# Autodesk Inventor assembly: arm_test
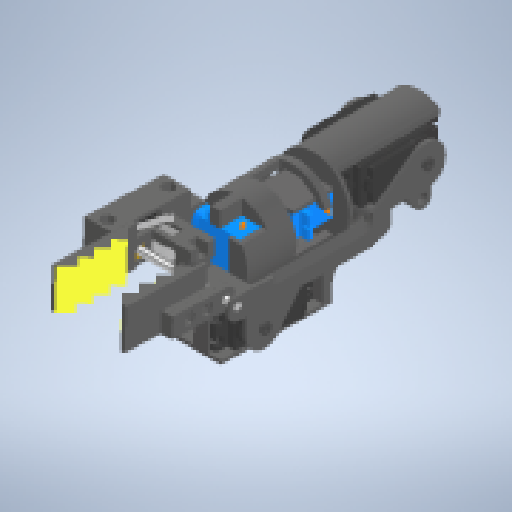
[picture p0: Inventor's stored thumbnail of the model, 512x512]
Saved by Autodesk Inventor 2024.1 (Build 281209000, 209)
## iProperties
Created: 2025-01-27
Part Number: arm_test
Document SubType Name: Assembly
Designer: hibik
Author: hibik
## Documents named in this file (15)
- C:\Users\hibik\Documents\Robomech\RESCUE\ORCA\hard\arm\arm_test.iam
- C:\Users\hibik\Documents\Robomech\RESCUE\ORCA\hard\arm\wrist_wrist.ipt
- C:\Users\hibik\Documents\Robomech\RESCUE\ORCA\hard\std_parts\Miusei_ms18.ipt
- C:\Users\hibik\Documents\Robomech\RESCUE\ORCA\hard\arm\wrist_geard_hone.ipt
- C:\Users\hibik\Documents\Robomech\RESCUE\ORCA\hard\arm\arm_2.ipt
- C:\Users\hibik\Documents\Robomech\RESCUE\ORCA\hard\std_parts\FS5103B.ipt
- C:\Users\hibik\Documents\Robomech\RESCUE\ORCA\hard\arm\arm_1.ipt
- C:\Users\hibik\Documents\Robomech\RESCUE\ORCA\hard\arm\hand_motor_setter_base.ipt
- C:\Users\hibik\Documents\Robomech\RESCUE\ORCA\hard\std_parts\motor_M4_55.ipt
- C:\Users\hibik\Documents\Robomech\RESCUE\ORCA\hard\std_parts\limit_switch.ipt
- C:\Users\hibik\Documents\Robomech\RESCUE\ORCA\hard\arm\hand_finger_inside.ipt
- C:\Users\hibik\Documents\Robomech\RESCUE\ORCA\hard\arm\hand_finger_outside.ipt
- C:\Users\hibik\Documents\Robomech\RESCUE\ORCA\hard\arm\hand_motor_setter_cover_under.ipt
- C:\Users\hibik\Documents\Robomech\RESCUE\ORCA\hard\arm\arm_0.ipt
- C:\Users\hibik\Documents\Robomech\RESCUE\ORCA\hard\arm\finger.ipt
## Components (17 placed, 14 different names)
1. wrist_wrist:1 — メイト:1, メイト:2, メイト:3, フラッシュ:2, メイト:4
2. Miusei_ms18:1 — メイト:1, メイト:2, メイト:3, フラッシュ:1, 挿入:3
3. Miusei_ms18:2 — 挿入:1, フラッシュ:1, フラッシュ:2, メイト:4, メイト:5, フラッシュ:3, フラッシュ:4
4. wrist_geard_hone:1 — 挿入:1
5. arm_2:1 — メイト:5, フラッシュ:3, フラッシュ:4, メイト:7, メイト:8, メイト:9
6. FS5103B:1 — メイト:7, メイト:8, 挿入:2, メイト:9
7. arm_1:1 — 挿入:2, 挿入:10
8. hand_motor_setter_base:1 — 挿入:3, 挿入:4, 角度:1, 挿入:5, 挿入:6, 角度:3, 角度:4, 挿入:8, 挿入:9, メイト:13, フラッシュ:5, メイト:14
9. motor_M4_55:1 — 挿入:4, 角度:1, 正接:1
10. limit_switch:1 — 挿入:5, 挿入:6
11. hand_finger_inside:1 — 挿入:7, 角度:2, 正接:1, 角度:4
12. hand_finger_outside:1 — 挿入:7, 角度:2, 角度:3, メイト:15
13. hand_motor_setter_cover_under:1 — 挿入:8, 挿入:9
14. arm_0:1 — メイト:10, メイト:11, メイト:12
15. FS5103B:2 — メイト:10, メイト:11, メイト:12, 挿入:10
16. finger:1 — メイト:13, フラッシュ:5, メイト:14, フラッシュ:6, フラッシュ:7
17. finger:2 — メイト:15, フラッシュ:6, フラッシュ:7
## Relationships (36: Mate 14, Insert 10, Flush 7, Angle 4, Tangent 1)
- メイト:1 [Mate]: wrist_wrist:1 ↔ Miusei_ms18:1
- メイト:2 [Mate]: wrist_wrist:1 ↔ Miusei_ms18:1
- メイト:3 [Mate] (0.1 mm): wrist_wrist:1 ↔ Miusei_ms18:1
- 挿入:1 [Insert]: Miusei_ms18:2 ↔ wrist_geard_hone:1
- フラッシュ:1 [Flush] (5.15 mm): Miusei_ms18:1 ↔ Miusei_ms18:2
- フラッシュ:2 [Flush] (-8 mm): wrist_wrist:1 ↔ Miusei_ms18:2
- メイト:4 [Mate] (2.4 mm): wrist_wrist:1 ↔ Miusei_ms18:2
- メイト:5 [Mate]: Miusei_ms18:2 ↔ arm_2:1
- フラッシュ:3 [Flush]: Miusei_ms18:2 ↔ arm_2:1
- フラッシュ:4 [Flush]: Miusei_ms18:2 ↔ arm_2:1
- メイト:7 [Mate]: arm_2:1 ↔ FS5103B:1
- メイト:8 [Mate]: arm_2:1 ↔ FS5103B:1
- 挿入:2 [Insert]: FS5103B:1 ↔ arm_1:1
- メイト:9 [Mate]: arm_2:1 ↔ FS5103B:1
- 挿入:3 [Insert]: Miusei_ms18:1 ↔ hand_motor_setter_base:1
- 挿入:4 [Insert] (0.1 mm): hand_motor_setter_base:1 ↔ motor_M4_55:1
- 角度:1 [Angle] (0 deg): hand_motor_setter_base:1 ↔ motor_M4_55:1
- 挿入:5 [Insert]: hand_motor_setter_base:1 ↔ limit_switch:1
- 挿入:6 [Insert]: hand_motor_setter_base:1 ↔ limit_switch:1
- 挿入:7 [Insert]: hand_finger_inside:1 ↔ hand_finger_outside:1
- 角度:2 [Angle] (180 deg): hand_finger_inside:1 ↔ hand_finger_outside:1
- 正接:1 [Tangent]: motor_M4_55:1 ↔ hand_finger_inside:1
- 角度:3 [Angle] (0 deg): hand_motor_setter_base:1 ↔ hand_finger_outside:1
- 角度:4 [Angle] (0 deg): hand_motor_setter_base:1 ↔ hand_finger_inside:1
- 挿入:8 [Insert]: hand_motor_setter_base:1 ↔ hand_motor_setter_cover_under:1
- 挿入:9 [Insert]: hand_motor_setter_base:1 ↔ hand_motor_setter_cover_under:1
- メイト:10 [Mate]: arm_0:1 ↔ FS5103B:2
- メイト:11 [Mate]: arm_0:1 ↔ FS5103B:2
- メイト:12 [Mate]: arm_0:1 ↔ FS5103B:2
- 挿入:10 [Insert]: arm_1:1 ↔ FS5103B:2
- メイト:13 [Mate]: hand_motor_setter_base:1 ↔ finger:1
- フラッシュ:5 [Flush]: hand_motor_setter_base:1 ↔ finger:1
- メイト:14 [Mate] (-25 mm): hand_motor_setter_base:1 ↔ finger:1
- メイト:15 [Mate]: hand_finger_outside:1 ↔ finger:2
- フラッシュ:6 [Flush]: finger:1 ↔ finger:2
- フラッシュ:7 [Flush]: finger:1 ↔ finger:2
